# Autodesk Inventor assembly: Drive Arm
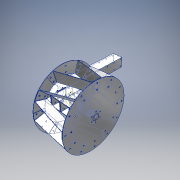
[picture p0: Inventor's stored thumbnail of the model, 180x180]
Saved by Autodesk Inventor 2019 (Build 230136000, 136)
## iProperties
Created: 2018-10-12
Part Number: Drive Arm
Document SubType Name: Assembly
Designer: Adhik
Mass: 2954.71 g
Surface Area: 9053.91 cm^2
Volume: 1103.34 cm^3
Density: 2.67797 g/cm^3
Author: Adhik
## Documents named in this file (11)
- I:\CAD\Julie\Drive Arm.iam
- I:\CAD\Julie\Arm 18 inch.ipt
- I:\CAD\Julie\Gearbox.iam
- I:\CAD\Julie\Arm 2 inch A.ipt
- I:\CAD\Julie\Arm 2 inch B.ipt
- I:\CAD\Julie\Arm 2 inch C.ipt
- I:\CAD\Julie\3775.ipt
- I:\CAD\Julie\Arm Bearing.ipt
- I:\CAD\Julie\Shaft.ipt
- I:\CAD\Julie\Wheel.iam
- I:\CAD\Julie\Shaft Coupler.ipt
## Components (11 placed, 10 different names)
1. Arm 18 inch:1 — Mate:1, Flush:1, Flush:2, Mate:3, Mate:16
2. Gearbox:1 [sub-assembly] — Mate:1, Mate:6, Mate:7, Mate:8, Mate:9, Mate:11
3. Arm 2 inch A:1 — Flush:1, Flush:2, Mate:3, Mate:4, Flush:4, Flush:5, Mate:6, Mate:7
4. Arm 2 inch B:1 — Mate:4, Mate:5, Flush:3, Flush:4, Flush:5, Flush:6
5. Arm 2 inch C:1 — Mate:5, Flush:3, Flush:6, Insert:1, Insert:2
6. 3775:1 — Mate:8, Mate:9, Mate:16
7. Arm Bearing:1 — Insert:2, Mate:10, Mate:13
8. Arm Bearing:2 — Insert:1, Mate:15
9. Shaft:1 — Mate:10, Mate:11, Mate:12, Mate:14
10. Wheel:1 [sub-assembly] — Mate:12, Mate:13
11. Shaft Coupler:1 — Mate:14, Mate:15
## Relationships (23: Mate 15, Flush 6, Insert 2)
- Mate:1: Arm 18 inch:1 ↔ Gearbox:1
- Flush:1: Arm 18 inch:1 ↔ Arm 2 inch A:1
- Flush:2: Arm 18 inch:1 ↔ Arm 2 inch A:1
- Mate:3: Arm 18 inch:1 ↔ Arm 2 inch A:1
- Mate:4: Arm 2 inch A:1 ↔ Arm 2 inch B:1
- Mate:5: Arm 2 inch B:1 ↔ Arm 2 inch C:1
- Flush:3: Arm 2 inch B:1 ↔ Arm 2 inch C:1
- Flush:4: Arm 2 inch A:1 ↔ Arm 2 inch B:1
- Flush:5: Arm 2 inch A:1 ↔ Arm 2 inch B:1
- Flush:6: Arm 2 inch B:1 ↔ Arm 2 inch C:1
- Mate:6: Gearbox:1 ↔ Arm 2 inch A:1
- Mate:7: Gearbox:1 ↔ Arm 2 inch A:1
- Mate:8: Gearbox:1 ↔ 3775:1
- Mate:9: Gearbox:1 ↔ 3775:1
- Insert:1: Arm 2 inch C:1 ↔ Arm Bearing:2
- Insert:2: Arm 2 inch C:1 ↔ Arm Bearing:1
- Mate:10: Arm Bearing:1 ↔ Shaft:1
- Mate:11: Gearbox:1 ↔ Shaft:1
- Mate:12: Shaft:1 ↔ Wheel:1
- Mate:13: Arm Bearing:1 ↔ Wheel:1
- Mate:14: Shaft:1 ↔ Shaft Coupler:1
- Mate:15: Arm Bearing:2 ↔ Shaft Coupler:1
- Mate:16: Arm 18 inch:1 ↔ 3775:1
